# Autodesk Inventor assembly: TR2 Visual Assembly
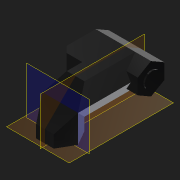
[picture p0: Inventor's stored thumbnail of the model, 180x180]
Saved by Autodesk Inventor 2017 (Build 210142000, 142)
## iProperties
Created: 2019-08-03
Part Number: TR2 Visual Assembly
Document SubType Name: Assembly
Designer: Dell
Author: Dell
## Documents named in this file (2)
- C:\Users\Dell\Documents\GitHub\tr2_essentials\tr2_description\meshes\Visual Assembly\link_a0.iam
- C:\Users\Dell\Documents\GitHub\tr2_essentials\tr2_description\meshes\Visual Assembly\link_a0.ipt
## Components (1 placed, 1 different names)
1. link_a0:1 — Mate:1, Mate:2, Mate:3
## Relationships (3: Mate 3)
- Mate:1: link_a0:1
- Mate:2: link_a0:1
- Mate:3: link_a0:1
